# Autodesk Inventor assembly: ThumbL3
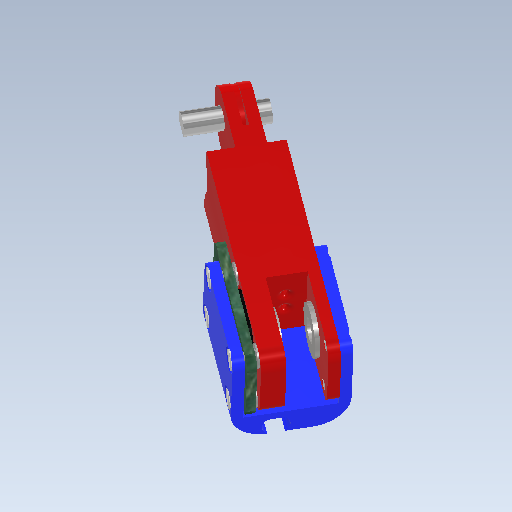
[picture p0: Inventor's stored thumbnail of the model, 512x512]
Saved by Autodesk Inventor 2020 (Build 240168000, 168)
## iProperties
Created: 2020-04-30
Part Number: ThumbL3
Document SubType Name: Assembly
Designer: sami_
Author: sami_
## Documents named in this file (10)
- C:\Users\sami_\Documents\V1.6\ThumbL3.iam
- C:\Users\sami_\Documents\V1.6\Workgroups\NotInProject\THUMB\Assembly\Thumblink.ipt
- C:\Users\sami_\Documents\V1.6\Workgroups\NotInProject\THUMB\Assembly\PotentiometerAssembly.iam
- C:\Users\sami_\Documents\V1.6\Libraries\Content Center Files\en-US\ISO 7089\ISO 7089 - 4 - 140 HV(1).ipt
- C:\Users\sami_\Documents\V1.6\Libraries\Content Center Files\en-US\ISO 1224-1 M\ISO 1224-1 - 17 - 4 x 7 x 2.ipt
- C:\Users\sami_\Documents\V1.6\Libraries\Content Center Files\en-US\ISO 7089\ISO 7089 - 1.6 - 140 HV(1).ipt
- C:\Users\sami_\Documents\V1.6\Workgroups\NotInProject\SHAFT.ipt
- C:\Users\sami_\Documents\V1.6\Workgroups\NotInProject\fingerpanel.ipt
- C:\Users\sami_\Documents\Inventor\Content Center Files\R2020\en-US\AS 1427(03)\AS 1427 - M2 x 8(1).ipt
- C:\Users\sami_\Documents\Inventor\Content Center Files\R2020\en-US\AS 1427(03)\AS 1427 - M2 x 4(1).ipt
## Components (20 placed, 9 different names)
1. Thumblink:1
2. PotentiometerAssembly:1 [sub-assembly]
3. ISO 7089 4:1
4. ISO 7089 4:2
5. ISO 1224-1 (Metric) 17 - 4 x 7 x 2:1
6. ISO 1224-1 (Metric) 17 - 4 x 7 x 2:2
7. ISO 7089 1.6:1
8. ISO 7089 1.6:2
9. ISO 7089 1.6:3
10. ISO 7089 1.6:4
11. SHAFT:1
12. fingerpanel:1 — Mate:6, Mate:7, Mate:8, Mate:9, Mate:10, Mate:11, Mate:12, Mate:13
13. AS 1427 - Metric M2 x 8:1 — Mate:6
14. AS 1427 - Metric M2 x 8:2 — Mate:7
15. AS 1427 - Metric M2 x 8:3 — Mate:8
16. AS 1427 - Metric M2 x 8:4 — Mate:9
17. AS 1427 - Metric M2 x 4:1 — Mate:10
18. AS 1427 - Metric M2 x 4:2 — Mate:11
19. AS 1427 - Metric M2 x 4:3 — Mate:12
20. AS 1427 - Metric M2 x 4:4 — Mate:13
## Relationships (22: Mate 13, WeldJoint 9)
- [Mate]: Thumblink:1 ↔ PotentiometerAssembly:1
- [Mate]: Thumblink:1 ↔ PotentiometerAssembly:1
- [WeldJoint]: ISO 7089 4:2 ↔ ISO 1224-1 (Metric) 17 - 4 x 7 x 2:2
- [WeldJoint]: ISO 7089 4:1 ↔ ISO 1224-1 (Metric) 17 - 4 x 7 x 2:1
- [WeldJoint]: Thumblink:1 ↔ ISO 7089 1.6:1
- [WeldJoint]: Thumblink:1 ↔ ISO 7089 1.6:2
- [WeldJoint]: Thumblink:1 ↔ ISO 7089 1.6:4
- [WeldJoint]: Thumblink:1 ↔ ISO 7089 1.6:3
- [Mate] (0.3 mm): PotentiometerAssembly:1 ↔ ISO 7089 1.6:1
- [WeldJoint]: Thumblink:1 ↔ ISO 7089 4:1
- [WeldJoint]: Thumblink:1 ↔ ISO 7089 4:2
- [Mate]: Thumblink:1 ↔ SHAFT:1
- [Mate]: Thumblink:1 ↔ SHAFT:1
- [WeldJoint]: Thumblink:1 ↔ fingerpanel:1
- Mate:6: fingerpanel:1 ↔ AS 1427 - Metric M2 x 8:1
- Mate:7: fingerpanel:1 ↔ AS 1427 - Metric M2 x 8:2
- Mate:8: fingerpanel:1 ↔ AS 1427 - Metric M2 x 8:3
- Mate:9: fingerpanel:1 ↔ AS 1427 - Metric M2 x 8:4
- Mate:10: fingerpanel:1 ↔ AS 1427 - Metric M2 x 4:1
- Mate:11: fingerpanel:1 ↔ AS 1427 - Metric M2 x 4:2
- Mate:12: fingerpanel:1 ↔ AS 1427 - Metric M2 x 4:3
- Mate:13: fingerpanel:1 ↔ AS 1427 - Metric M2 x 4:4
